# Autodesk Inventor assembly: 002_Bo_truot
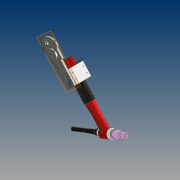
[picture p0: Inventor's stored thumbnail of the model, 180x180]
Saved by Autodesk Inventor 2021 (Build 250183000, 183)
## iProperties
Created: 2024-04-05
Part Number: 002_Bo_truot
Document SubType Name: Assembly
Designer: Admin
Author: Admin
## Documents named in this file (5)
- C:\Users\Admin\Desktop\DO_AN_TOT_NGHIEP_2024\Mechanical\Design_in_3D\Version_1\002_Bo_truot.iam
- C:\Users\Admin\Desktop\DO_AN_TOT_NGHIEP_2024\Mechanical\Design_in_3D\Version_1\17_Khau_noi_tiep_cuoi.ipt
- C:\Users\Admin\Desktop\DO_AN_TOT_NGHIEP_2024\Mechanical\Design_in_3D\Version_1\18_Kep_han_A.ipt
- C:\Users\Admin\Desktop\Do_an\Ver_3\TIG GUN_2.ipt
- C:\Users\Admin\Desktop\DO_AN_TOT_NGHIEP_2024\Mechanical\Design_in_3D\Version_1\19_Kep_han_B.ipt
## Components (4 placed, 4 different names)
1. 17_Khau_noi_tiep_cuoi:1 — Flush:1, Flush:2, Angle:1, Mate:11
2. 18_Kep_han_A:1 — Flush:1, Flush:2, Mate:8, Angle:2, Flush:3, Mate:11
3. TIG GUN_2:1 — Mate:8, Angle:1, Mate:10, Flush:4
4. 19_Kep_han_B:1 — Mate:10, Angle:2, Flush:3, Flush:4
## Relationships (9: Flush 4, Mate 3, Angle 2)
- Flush:1: 17_Khau_noi_tiep_cuoi:1 ↔ 18_Kep_han_A:1
- Flush:2: 17_Khau_noi_tiep_cuoi:1 ↔ 18_Kep_han_A:1
- Mate:8: 18_Kep_han_A:1 ↔ TIG GUN_2:1
- Angle:1 (0 deg): 17_Khau_noi_tiep_cuoi:1 ↔ TIG GUN_2:1
- Mate:10: TIG GUN_2:1 ↔ 19_Kep_han_B:1
- Angle:2 (0 deg): 18_Kep_han_A:1 ↔ 19_Kep_han_B:1
- Flush:3: 18_Kep_han_A:1 ↔ 19_Kep_han_B:1
- Flush:4 (-30 mm): TIG GUN_2:1 ↔ 19_Kep_han_B:1
- Mate:11: 17_Khau_noi_tiep_cuoi:1 ↔ 18_Kep_han_A:1
